# Autodesk Inventor assembly: NewBeltGear
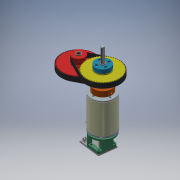
[picture p0: Inventor's stored thumbnail of the model, 180x180]
Saved by Autodesk Inventor 2019.1 (Build 231200000, 200)
## iProperties
Created: 2018-08-27
Part Number: NewBeltGear
Material: Generisch
Document SubType Name: Assembly
Designer: JochenAlt
Author: JochenAlt
## Documents named in this file (13)
- D:\Projects\Ondine\CAD\Beltdrive\BeltGear.iam
- D:\Projects\Ondine\CAD\Beltdrive\Construction\Input.ipt
- D:\Projects\Ondine\CAD\Beltdrive\Construction\Output.ipt
- D:\Projects\Ondine\CAD\Beltdrive\Construction\BeltGear.ipt
- D:\Projects\Ondine\CAD\Beltdrive\Construction\Zahnriemen4.ipt
- D:\Projects\Ondine\CAD\Mounting Hub.ipt
- D:\Projects\Ondine\CAD\Bearings\AST_Bearings_SMR74.ipt
- D:\Projects\Ondine\CAD\HarmonicDrive-Axis.ipt
- D:\Projects\Ondine\CAD\Motor.iam
- C:\Users\JochenAlt\Documents\Inventor\Content Center Files\R2019\de-DE\BS 4168(5)\BS 4168 - M3 x 6(5).ipt
- C:\Users\JochenAlt\Documents\Inventor\Content Center Files\R2019\de-DE\DIN 912\DIN 912 - M3 x 0,5 x 8 x 6,75.ipt
- D:\Projects\Ondine\CAD\Encoder\MagneticEncoder.iam
- D:\Projects\Ondine\CAD\BushBeltDriveTL.ipt
## Components (20 placed, 12 different names)
1. Input:1 — Passend:1, Passend:13, Passend:17, Passend:18, Drehung:1, Drehung:2, Passend:26
2. output:1 — Passend:8, Passend:15, Einfügen:1, Einfügen:2, Einfügen:3, Einfügen:4, Drehung:4, Passend:25, Fluchtend:2, Drehung:5
3. beltGeaR:1 — Passend:9, Passend:10, Fluchtend:1, Drehung:2, Passend:26, Fluchtend:2, Drehung:5, Passend:44, Passend:45
4. Zahnriemen:1 — Passend:5, Passend:6, Passend:7, Passend:8, Passend:12, Passend:14, Passend:23
5. Zahnriemen:2 — Passend:4, Passend:7, Passend:10, Fluchtend:1, Passend:34
6. Mounting Hub:1 — Passend:12, Passend:13, Drehung:1, Passend:22, Passend:30, Passend:31, Passend:32
7. Mounting Hub:2 — Passend:14, Passend:15, Drehung:4, Passend:28, Passend:35, Passend:37, Passend:43
8. DIN 912 - ersetzt durch DIN EN ISO 4762 M3 x 8:2 — Einfügen:1
9. DIN 912 - ersetzt durch DIN EN ISO 4762 M3 x 8:4 — Einfügen:2
10. DIN 912 - ersetzt durch DIN EN ISO 4762 M3 x 8:1 — Einfügen:3
11. DIN 912 - ersetzt durch DIN EN ISO 4762 M3 x 8:3 — Einfügen:4, Passend:37
12. AST_Bearings_SMR74:1 — Passend:25, Passend:38
13. AST_Bearings_SMR74:2 — Passend:17, Passend:18, Passend:33
14. HarmonicDrive-Axis:1 — Passend:28, Passend:33, Passend:36, Passend:38, Passend:42
15. Motor:1 [sub-assembly] — Passend:31, Passend:32, Passend:39, Passend:40, Passend:41
16. BS 4168 : Teil 5 Innensechskantschrauben und Stiftschlüssel, metrische Ausführung - Spezifikation für Sechskant-Gewindestifte mit Ringschneide - Metrisch M3 x 6:2 — Passend:30, Passend:34
17. BS 4168 : Teil 5 Innensechskantschrauben und Stiftschlüssel, metrische Ausführung - Spezifikation für Sechskant-Gewindestifte mit Ringschneide - Metrisch M3 x 6:1 — Passend:35, Passend:36
18. EncoderedMotor:1 [sub-assembly] — Passend:39, Passend:40, Passend:41
19. BushOmniWheel:1 — Passend:42, Passend:43
20. BushOmniWheel:2 — Passend:44, Passend:45
## Relationships (45: Mate 35, Insert 4, RelateRotation 4, Flush 2)
- Passend:1 [Mate]: Input:1
- Passend:4 [Mate]: Zahnriemen:2
- Passend:5 [Mate]: Zahnriemen:1
- Passend:6 [Mate]: Zahnriemen:1
- Passend:7 [Mate]: Zahnriemen:1 ↔ Zahnriemen:2
- Passend:8 [Mate]: output:1 ↔ Zahnriemen:1
- Passend:9 [Mate]: beltGeaR:1
- Passend:10 [Mate] (31.3 mm): beltGeaR:1 ↔ Zahnriemen:2
- Fluchtend:1 [Flush] (0.5 mm): beltGeaR:1 ↔ Zahnriemen:2
- Passend:12 [Mate]: Zahnriemen:1 ↔ Mounting Hub:1
- Passend:13 [Mate]: Input:1 ↔ Mounting Hub:1
- Passend:14 [Mate]: Zahnriemen:1 ↔ Mounting Hub:2
- Passend:15 [Mate]: output:1 ↔ Mounting Hub:2
- Einfügen:1 [Insert]: output:1 ↔ DIN 912 - ersetzt durch DIN EN ISO 4762 M3 x 8:2
- Einfügen:2 [Insert]: output:1 ↔ DIN 912 - ersetzt durch DIN EN ISO 4762 M3 x 8:4
- Einfügen:3 [Insert]: output:1 ↔ DIN 912 - ersetzt durch DIN EN ISO 4762 M3 x 8:1
- Einfügen:4 [Insert]: output:1 ↔ DIN 912 - ersetzt durch DIN EN ISO 4762 M3 x 8:3
- Passend:17 [Mate]: Input:1 ↔ AST_Bearings_SMR74:2
- Passend:18 [Mate]: Input:1 ↔ AST_Bearings_SMR74:2
- Drehung:1 [RelateRotation] (1 ul): Input:1 ↔ Mounting Hub:1
- Drehung:2 [RelateRotation] (0.3333 ul): Input:1 ↔ beltGeaR:1
- Drehung:4 [RelateRotation] (1 ul): output:1 ↔ Mounting Hub:2
- Passend:22 [Mate]: Mounting Hub:1
- Passend:23 [Mate]: Zahnriemen:1
- Passend:25 [Mate]: output:1 ↔ AST_Bearings_SMR74:1
- Passend:26 [Mate] (1.15 mm): Input:1 ↔ beltGeaR:1
- Fluchtend:2 [Flush] (1.35 mm): output:1 ↔ beltGeaR:1
- Drehung:5 [RelateRotation] (0.3333 ul): output:1 ↔ beltGeaR:1
- Passend:28 [Mate]: Mounting Hub:2 ↔ HarmonicDrive-Axis:1
- Passend:30 [Mate]: Mounting Hub:1 ↔ BS 4168 : Teil 5 Innensechskantschrauben und Stiftschlüssel, metrische Ausführung - Spezifikation für Sechskant-Gewindestifte mit Ringschneide - Metrisch M3 x 6:2
- Passend:31 [Mate]: Mounting Hub:1 ↔ Motor:1
- Passend:32 [Mate] (0.5 mm): Mounting Hub:1 ↔ Motor:1
- Passend:33 [Mate]: AST_Bearings_SMR74:2 ↔ HarmonicDrive-Axis:1
- Passend:34 [Mate] (2 mm): Zahnriemen:2 ↔ BS 4168 : Teil 5 Innensechskantschrauben und Stiftschlüssel, metrische Ausführung - Spezifikation für Sechskant-Gewindestifte mit Ringschneide - Metrisch M3 x 6:2
- Passend:35 [Mate]: Mounting Hub:2 ↔ BS 4168 : Teil 5 Innensechskantschrauben und Stiftschlüssel, metrische Ausführung - Spezifikation für Sechskant-Gewindestifte mit Ringschneide - Metrisch M3 x 6:1
- Passend:36 [Mate] (2 mm): HarmonicDrive-Axis:1 ↔ BS 4168 : Teil 5 Innensechskantschrauben und Stiftschlüssel, metrische Ausführung - Spezifikation für Sechskant-Gewindestifte mit Ringschneide - Metrisch M3 x 6:1
- Passend:37 [Mate]: Mounting Hub:2 ↔ DIN 912 - ersetzt durch DIN EN ISO 4762 M3 x 8:3
- Passend:38 [Mate]: AST_Bearings_SMR74:1 ↔ HarmonicDrive-Axis:1
- Passend:39 [Mate]: Motor:1 ↔ EncoderedMotor:1
- Passend:40 [Mate]: Motor:1 ↔ EncoderedMotor:1
- Passend:41 [Mate]: Motor:1 ↔ EncoderedMotor:1
- Passend:42 [Mate]: HarmonicDrive-Axis:1 ↔ BushOmniWheel:1
- Passend:43 [Mate]: Mounting Hub:2 ↔ BushOmniWheel:1
- Passend:44 [Mate]: beltGeaR:1 ↔ BushOmniWheel:2
- Passend:45 [Mate]: beltGeaR:1 ↔ BushOmniWheel:2
